# Autodesk Inventor assembly: Subensamble_Base cortadora_MIR
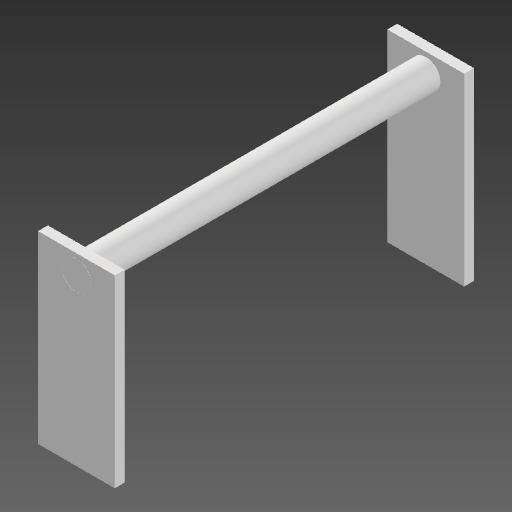
[picture p0: Inventor's stored thumbnail of the model, 512x512]
Saved by Autodesk Inventor 2021 (Build 250183000, 183)
## iProperties
Created: 2021-04-30
Part Number: Subensamble_Base cortadora_MIR
Document SubType Name: Assembly
Designer: maaro
Author: Admin
## Documents named in this file (3)
- C:\Users\maaro\Documents\UNAL\Automatización de Procesos de Manufactura\Github\Proyecto_APM\CADs estaciones a automatizar\Estación corte\Subensamble_Base cortadora_MIR.iam
- C:\Users\maaro\Documents\UNAL\Automatización de Procesos de Manufactura\Github\Proyecto_APM\CADs estaciones a automatizar\Estación corte\Base_cortadora_MIR.ipt
- C:\Users\maaro\Documents\UNAL\Automatización de Procesos de Manufactura\Github\Proyecto_APM\CADs estaciones a automatizar\Estación corte\Barra base cotadora_MIR.ipt
## Components (3 placed, 2 different names)
1. Base_cortadora_MIR:1 — Flush:1, Rotational:1
2. Base_cortadora_MIR:2 — Flush:2, Mate:1
3. Barra base cotadora_MIR:1 — Flush:2, Mate:1, Flush:1, Rotational:1
## Relationships (4: Flush 2, Mate 1, RevoluteJoint 1)
- Flush:2: Base_cortadora_MIR:2 ↔ Barra base cotadora_MIR:1
- Mate:1: Base_cortadora_MIR:2 ↔ Barra base cotadora_MIR:1
- Flush:1: Base_cortadora_MIR:1 ↔ Barra base cotadora_MIR:1
- Rotational:1 [RevoluteJoint]: Base_cortadora_MIR:1 ↔ Barra base cotadora_MIR:1
